# Autodesk Inventor assembly: DBK_42ToothPulley V2
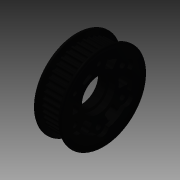
[picture p0: Inventor's stored thumbnail of the model, 180x180]
Saved by Autodesk Inventor 2014 SP1 (Build 180222100, 222)
## iProperties
Created: 2013-01-12
Part Number: DBK_42ToothPulley V2
Document SubType Name: Assembly
Designer: Moses
Mass: 50.695 g
Surface Area: 261.005 cm^2
Volume: 42.2458 cm^3
Density: 1.2 g/cm^3
Author: Moses
## Documents named in this file (2)
- C:\Users\Moses\Documents\Inventor\Sally Rebuild\Rebuild Sally\DBK_42ToothPulley V2.iam
- C:\Users\Moses\Documents\Inventor\Sally Rebuild\Rebuild Sally\DBK_42ToothPulleyHalf_am-2234-half.ipt
## Components (2 placed, 1 different names)
1. DBK_42ToothPulleyHalf_am-2234-half:1 — Insert:8, Mate:1
2. DBK_42ToothPulleyHalf_am-2234-half:2 — Insert:8, Mate:1
## Relationships (2: Insert 1, Mate 1)
- Insert:8: DBK_42ToothPulleyHalf_am-2234-half:1 ↔ DBK_42ToothPulleyHalf_am-2234-half:2
- Mate:1: DBK_42ToothPulleyHalf_am-2234-half:1 ↔ DBK_42ToothPulleyHalf_am-2234-half:2
